# Autodesk Inventor assembly: Churrasqueira
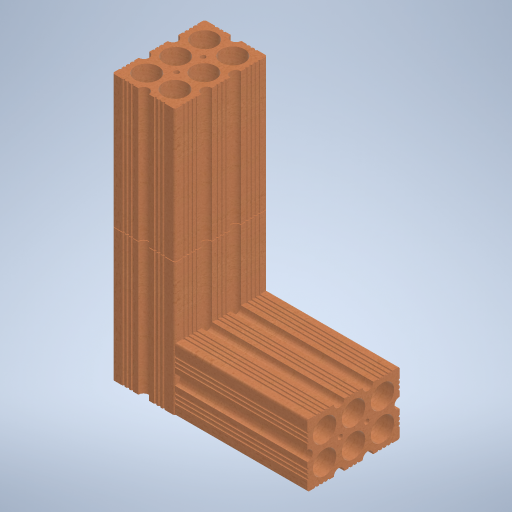
[picture p0: Inventor's stored thumbnail of the model, 512x512]
Saved by Autodesk Inventor 2024.4 (Build 284460000, 460)
## iProperties
Created: 2026-08-29
Part Number: Churrasqueira
Document SubType Name: Assembly
Designer: MaryPinkAssus
Author: MaryPinkAssus
## Documents named in this file (2)
- C:\Users\MaryPinkAssus\Documents\Inventor\Churas\Churrasqueira.iam
- C:\Users\MaryPinkAssus\Documents\Inventor\Churas\Tijolo 9x19cm.ipt
## Components (3 placed, 1 different names)
1. Tijolo 9x19cm:1 — Mate:1, Mate:2, Flush:1, Mate:3, Flush:2, Flush:3, Mate:4, Flush:4, Flush:5
2. Tijolo 9x19cm:2 — Mate:3, Flush:2, Flush:3
3. Tijolo 9x19cm:3 — Mate:4, Flush:4, Flush:5
## Relationships (9: Flush 5, Mate 4)
- Mate:1: Tijolo 9x19cm:1
- Mate:2: Tijolo 9x19cm:1
- Flush:1: Tijolo 9x19cm:1
- Mate:3 (1 mm): Tijolo 9x19cm:1 ↔ Tijolo 9x19cm:2
- Flush:2: Tijolo 9x19cm:1 ↔ Tijolo 9x19cm:2
- Flush:3: Tijolo 9x19cm:1 ↔ Tijolo 9x19cm:2
- Mate:4: Tijolo 9x19cm:1 ↔ Tijolo 9x19cm:3
- Flush:4: Tijolo 9x19cm:1 ↔ Tijolo 9x19cm:3
- Flush:5: Tijolo 9x19cm:1 ↔ Tijolo 9x19cm:3
